# Autodesk Inventor assembly: Zmotionassembly
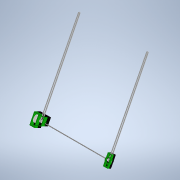
[picture p0: Inventor's stored thumbnail of the model, 180x180]
Saved by Autodesk Inventor 2020.4 (Build 244396000, 396)
## iProperties
Created: 2021-03-29
Part Number: Zmotionassembly
Document SubType Name: Assembly
Designer: AOB
Mass: 266.326 g
Surface Area: 1026.66 cm^2
Volume: 151.373 cm^3
Density: 1.7594 g/cm^3
Author: AOB
## Documents named in this file (5)
- C:\Users\marti\Documents\Inventor\ProjectBoron\Boron Ultima\Zmotionassembly.iam
- C:\Users\marti\Documents\Inventor\ProjectBoron\Boron Ultima\Z-powertrain.iam
- C:\Users\marti\Documents\Inventor\ProjectBoron\Boron Ultima\bottom idler housing.iam
- C:\Users\marti\Documents\Inventor\ProjectBoron\Boron Ultima\zmotorblock.iam
- C:\Users\marti\Documents\Inventor\ProjectBoron\Boron Ultima\z-belt.ipt
## Components (5 placed, 4 different names)
1. Z-powertrain:1 [sub-assembly] — Mate:2, Flush:1, Mate:3, Flush:2, Rotational:2, Rotational:3
2. bottom idler housing:1 [sub-assembly] — Mate:2, Flush:1, Angle:1
3. zmotorblock:1 [sub-assembly] — Mate:3, Flush:2, Angle:2
4. z-belt:1 — Rotational:2, Angle:1, Angle:3
5. z-belt:2 — Rotational:3, Angle:2, Angle:3
## Relationships (9: Angle 3, Mate 2, Flush 2, RevoluteJoint 2)
- Mate:2: Z-powertrain:1 ↔ bottom idler housing:1
- Flush:1: Z-powertrain:1 ↔ bottom idler housing:1
- Mate:3: Z-powertrain:1 ↔ zmotorblock:1
- Flush:2: Z-powertrain:1 ↔ zmotorblock:1
- Rotational:2 [RevoluteJoint] (0.5 mm): Z-powertrain:1 ↔ z-belt:1
- Rotational:3 [RevoluteJoint] (-0.9 mm): Z-powertrain:1 ↔ z-belt:2
- Angle:1 (180 deg): bottom idler housing:1 ↔ z-belt:1
- Angle:2 (180 deg): zmotorblock:1 ↔ z-belt:2
- Angle:3 (0 deg): z-belt:1 ↔ z-belt:2
